# Autodesk Inventor assembly: main assembly
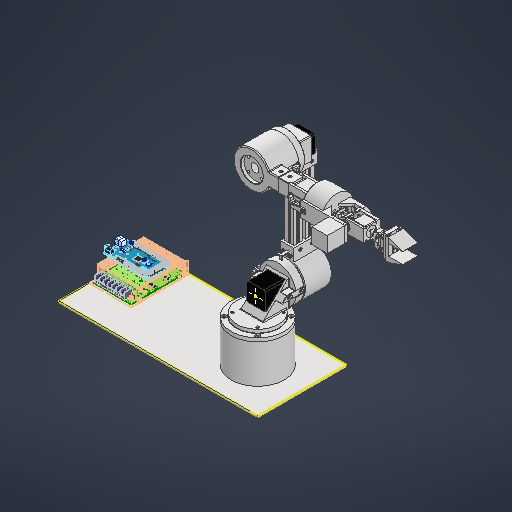
[picture p0: Inventor's stored thumbnail of the model, 512x512]
Saved by Autodesk Inventor 2026.2 (Build 302298000, 298)
## iProperties
Created: 2025-07-04
Part Number: main assembly
Document SubType Name: Assembly
Designer: gavin
Author: gavin
## Documents named in this file (38)
- D:\Github\6-DOF-Robot-Arm\3D-model\robot armT 2(CAD file)\main assembly.iam
- D:\Github\6-DOF-Robot-Arm\3D-model\robot armT 2(CAD file)\stepper 42x48 - 27.ipt
- D:\Github\6-DOF-Robot-Arm\3D-model\robot armT 2(CAD file)\28stepper27.ipt
- D:\Github\6-DOF-Robot-Arm\3D-model\robot armT 2(CAD file)\CSN 02 4630 - 6009.ipt
- D:\Github\6-DOF-Robot-Arm\3D-model\robot armT 2(CAD file)\CNS 2862 B2116 - 6007 - 35 x 62 x 14.ipt
- D:\Github\6-DOF-Robot-Arm\3D-model\robot armT 2(CAD file)\base plate.ipt
- D:\Github\6-DOF-Robot-Arm\3D-model\robot armT 2(CAD file)\stepper 42x60 -50 .ipt
- D:\Github\6-DOF-Robot-Arm\3D-model\robot armT 2(CAD file)\j2 42 motor mount.ipt
- D:\Github\6-DOF-Robot-Arm\3D-model\robot armT 2(CAD file)\j1 assmble.iam
- D:\Github\6-DOF-Robot-Arm\3D-model\robot armT 2(CAD file)\optic endstop module.ipt
- D:\Github\6-DOF-Robot-Arm\3D-model\robot armT 2(CAD file)\j2j3 alumi ext.ipt
- D:\Github\6-DOF-Robot-Arm\3D-model\robot armT 2(CAD file)\j3 motor mount.ipt
- D:\Github\6-DOF-Robot-Arm\3D-model\robot armT 2(CAD file)\j3j4 alumi ext.ipt
- D:\Github\6-DOF-Robot-Arm\3D-model\robot armT 2(CAD file)\j2 endstop blocker.ipt
- D:\Github\6-DOF-Robot-Arm\3D-model\robot armT 2(CAD file)\j3 endstop blocker.ipt
- D:\Github\6-DOF-Robot-Arm\3D-model\robot armT 2(CAD file)\6mm axle hub.ipt
- D:\Github\6-DOF-Robot-Arm\3D-model\robot armT 2(CAD file)\j4 motor mount.ipt
- D:\Github\6-DOF-Robot-Arm\3D-model\robot armT 2(CAD file)\j4 motor mount cover.ipt
- D:\Github\6-DOF-Robot-Arm\3D-model\robot armT 2(CAD file)\j4 moving part.ipt
- D:\Github\6-DOF-Robot-Arm\3D-model\robot armT 2(CAD file)\nema 11x25.ipt
- D:\Github\6-DOF-Robot-Arm\3D-model\robot armT 2(CAD file)\5mm axle hub.ipt
- D:\Github\6-DOF-Robot-Arm\3D-model\robot armT 2(CAD file)\bearing 22-M6.ipt
- D:\Github\6-DOF-Robot-Arm\3D-model\robot armT 2(CAD file)\j6 motor mount v2.ipt
- D:\Github\6-DOF-Robot-Arm\3D-model\robot armT 2(CAD file)\j4 endstop blocker.ipt
- D:\Github\6-DOF-Robot-Arm\3D-model\robot armT 2(CAD file)\sg90 long claw.iam
- D:\Github\6-DOF-Robot-Arm\3D-model\robot armT 2(CAD file)\35x40 stepper.ipt
- D:\Github\6-DOF-Robot-Arm\3D-model\robot armT 2(CAD file)\j3 moving part option3.ipt
- D:\Github\6-DOF-Robot-Arm\3D-model\robot armT 2(CAD file)\z21 8x18.ipt
- D:\Github\6-DOF-Robot-Arm\3D-model\robot armT 2(CAD file)\18mm hub.ipt
- D:\Github\6-DOF-Robot-Arm\3D-model\robot armT 2(CAD file)\j2 moving part option2.ipt
- D:\Github\6-DOF-Robot-Arm\3D-model\robot armT 2(CAD file)\M5 heat set inserts.ipt
- D:\Github\6-DOF-Robot-Arm\3D-model\robot armT 2(CAD file)\AS 1427 - M3 x 6(5) II.ipt
- D:\Github\6-DOF-Robot-Arm\3D-model\robot armT 2(CAD file)\M3 heat set insert.ipt
- D:\Github\6-DOF-Robot-Arm\3D-model\robot armT 2(CAD file)\CNS 4557 - M4 x 0.7 x 10.ipt
- D:\Github\6-DOF-Robot-Arm\3D-model\robot armT 2(CAD file)\AS 1474 - M4(1).ipt
- D:\Github\6-DOF-Robot-Arm\3D-model\robot armT 2(CAD file)\AS 1474 - M3(1).ipt
- D:\Github\6-DOF-Robot-Arm\3D-model\robot armT 2(CAD file)\ArduinoMega2560\ArduinoMega2560\ArduinoMega2560.ipt
- D:\Github\6-DOF-Robot-Arm\3D-model\robot armT 2(CAD file)\VTX-212-100-0xx\VTX-212-100-0xx\VTX-212-100-0xx.ipt
## Components (101 placed, 37 different names)
1. base plate:1 — 齊平:5, 貼合:133, 齊平:22, 貼合:134
2. j1 assmble:1 [sub-assembly]
3. stepper 42x48 - 27:2 — 貼合:45, 貼合:46, 貼合:47, 貼合:110, 齊平:18
4. CSN 02 4630 - 6009:1 — 貼合:48, 貼合:49
5. CSN 02 4630 - 6009:2 — 貼合:16, 貼合:29
6. CNS 2862 B2116 - 6007 - 35 x 62 x 14:1 — 剛性:108, 剛性:109
7. stepper 42x60 -50 :1 — 貼合:16, 貼合:27, 貼合:28, 剛性:106
8. j2 42 motor mount:1 — 貼合:27, 貼合:28, 貼合:29, 貼合:33, 貼合:34, 貼合:35, 剛性:12, 剛性:13
9. optic endstop module:1 — 貼合:33, 貼合:34, 貼合:35, 齊平:10, 剛性:10, 剛性:11
10. j2j3 alumi ext:1 — 剛性:5, 剛性:7
11. j2j3 alumi ext:2 — 剛性:6
12. j3 motor mount:1 — 貼合:45, 貼合:46, 貼合:47, 貼合:48, 貼合:49, 齊平:11, 齊平:12, 貼合:59, 剛性:7, 貼合:132, 剛性:65, 剛性:66, 剛性:67, 剛性:68, 剛性:107
13. j3j4 alumi ext:1 — 剛性:4, 剛性:8
14. optic endstop module:2 — 貼合:129, 貼合:130, 貼合:131, 剛性:20, 剛性:21, 剛性:22, 剛性:23
15. j2 endstop blocker:1 — 齊平:10, 貼合:117, 貼合:118, 貼合:119, 剛性:14, 剛性:15, 剛性:16, 剛性:17
16. j3 endstop blocker:1 — 齊平:11, 齊平:12, 貼合:59, 貼合:132, 剛性:18, 剛性:19, 剛性:24, 剛性:25
17. 6mm axle hub:1 — 貼合:123, 貼合:124, 貼合:125
18. j4 motor mount:1 — 齊平:14, 齊平:15, 貼合:62, 貼合:65, 貼合:71, 貼合:72, 貼合:73, 齊平:21, 剛性:8, 剛性:9, 剛性:27, 剛性:28, 剛性:72, 剛性:75, 剛性:108
19. j4 motor mount cover:1 — 齊平:14, 齊平:15, 貼合:62, 貼合:65
20. 28stepper27:1 — 剛性:9
21. optic endstop module:3 — 貼合:71, 貼合:72, 貼合:73, 剛性:29, 剛性:30
22. j4 moving part:1 — 貼合:74, 貼合:76, 貼合:86, 貼合:87, 貼合:104, 貼合:105, 貼合:107, 貼合:108, 貼合:109, 貼合:123, 貼合:124, 貼合:125, 貼合:126, 貼合:127, 剛性:26, 剛性:32, 剛性:33, 剛性:109
23. nema 11x25:1 — 貼合:88, 貼合:89, 貼合:103, 貼合:128, 剛性:111
24. optic endstop module:4 — 貼合:74, 貼合:76, 貼合:107, 剛性:34, 剛性:35
25. 5mm axle hub:1 — 剛性:1, 剛性:110
26. bearing 22-M6:1 — 貼合:86, 貼合:87
27. j6 motor mount v2:1 — 貼合:88, 貼合:89, 貼合:128, 剛性:110
28. j4 endstop blocker:1 — 貼合:108, 貼合:109, 貼合:126, 剛性:31
29. sg90 long claw:1 [sub-assembly] — 貼合:99, 貼合:100, 貼合:103
30. 5mm axle hub:2 — 貼合:99, 貼合:100, 剛性:111
31. 35x40 stepper:1 — 貼合:104, 貼合:105, 剛性:1, 貼合:127
32. j3 moving part option3:1 — 剛性:4, 貼合:120, 貼合:121, 貼合:122, 齊平:21, 貼合:129, 貼合:130, 貼合:131, 剛性:40, 剛性:41, 剛性:42, 剛性:43, 剛性:73, 剛性:74, 剛性:107
33. z21 8x18:1 — 貼合:110, 齊平:18
34. 18mm hub:1 — 貼合:120, 貼合:121, 貼合:122
35. j2 moving part option2:1 — 剛性:5, 貼合:114, 貼合:115, 貼合:116, 貼合:117, 貼合:118, 貼合:119, 剛性:6, 剛性:36, 剛性:37, 剛性:38, 剛性:39, 剛性:59, 剛性:60, 剛性:61, 剛性:62
36. z21 8x18:2 — 剛性:105, 剛性:106
37. 18mm hub:2 — 剛性:105, 貼合:114, 貼合:115, 貼合:116
38. AS 1427 - M3 x 6(5) II:1 — 剛性:16
39. AS 1427 - M3 x 6(5) II:2 — 剛性:23
40. AS 1427 - M3 x 6(5) II:3 — 剛性:24
41. AS 1427 - M3 x 6(5) II:4 — 剛性:22
42. AS 1427 - M3 x 6(5) II:5 — 剛性:17
43. AS 1427 - M3 x 6(5) II:6 — 剛性:25
44. AS 1427 - M3 x 6(5) II:7 — 剛性:10
45. AS 1427 - M3 x 6(5) II:8 — 剛性:11
46. M3 heat set insert:1 — 剛性:15
47. M3 heat set insert:2 — 剛性:13
48. M3 heat set insert:3 — 剛性:26
49. M3 heat set insert:4 — 剛性:32
50. M3 heat set insert:5 — 剛性:28
51. M3 heat set insert:6 — 剛性:19
52. M3 heat set insert:7 — 剛性:20
53. M3 heat set insert:8 — 剛性:12
54. M3 heat set insert:9 — 剛性:14
55. M3 heat set insert:10 — 剛性:33
56. M3 heat set insert:14 — 剛性:27
57. M3 heat set insert:15 — 剛性:18
58. M3 heat set insert:18 — 剛性:21
59. AS 1427 - M3 x 6(5) II:9 — 剛性:29
60. AS 1427 - M3 x 6(5) II:10 — 剛性:35
61. AS 1427 - M3 x 6(5) II:11 — 剛性:31
62. AS 1427 - M3 x 6(5) II:12 — 剛性:30
63. AS 1427 - M3 x 6(5) II:13 — 剛性:34
64. M5 heat set inserts:5 — 剛性:39
65. M5 heat set inserts:6 — 剛性:36
66. M5 heat set inserts:10 — 剛性:42
67. M5 heat set inserts:11 — 剛性:41
68. M5 heat set inserts:12 — 剛性:40
69. M5 heat set inserts:13 — 剛性:38
70. M5 heat set inserts:14 — 剛性:37
71. M5 heat set inserts:18 — 剛性:43
72. CNS 4557 - M4 x 0.7 x 10:1 — 剛性:64, 剛性:65
73. CNS 4557 - M4 x 0.7 x 10:2 — 剛性:57, 剛性:60
74. CNS 4557 - M4 x 0.7 x 10:3 — 剛性:55, 剛性:74
75. CNS 4557 - M4 x 0.7 x 10:4 — 剛性:53, 剛性:67
76. CNS 4557 - M4 x 0.7 x 10:5 — 剛性:58, 剛性:59
77. CNS 4557 - M4 x 0.7 x 10:6 — 剛性:56, 剛性:62
78. CNS 4557 - M4 x 0.7 x 10:7 — 剛性:54, 剛性:68
79. CNS 4557 - M4 x 0.7 x 10:8 — 剛性:52, 剛性:61
80. CNS 4557 - M4 x 0.7 x 10:9 — 剛性:71, 剛性:72
81. CNS 4557 - M4 x 0.7 x 10:10 — 剛性:70, 剛性:73
82. CNS 4557 - M4 x 0.7 x 10:11 — 剛性:63, 剛性:66
83. CNS 4557 - M4 x 0.7 x 10:12 — 剛性:69, 剛性:75
84. AS 1474 - M4(1):1 — 剛性:57
85. AS 1474 - M4(1):2 — 剛性:55
86. AS 1474 - M4(1):5 — 剛性:56
87. AS 1474 - M4(1):6 — 剛性:53
88. AS 1474 - M4(1):7 — 剛性:54
89. AS 1474 - M4(1):11 — 剛性:64
90. AS 1474 - M4(1):12 — 剛性:63
91. AS 1474 - M4(1):13 — 剛性:71
92. AS 1474 - M4(1):14 — 剛性:69
93. AS 1474 - M4(1):15 — 剛性:70
94. AS 1474 - M4(1):16 — 剛性:52
95. AS 1474 - M4(1):18 — 剛性:58
96. AS 1474 - M3(1):1
97. AS 1474 - M3(1):2
98. AS 1474 - M3(1):3
99. AS 1474 - M3(1):5
100. ArduinoMega2560:1
101. VTX-212-100-0xx:1 — 貼合:133, 齊平:22, 貼合:134
## Relationships (149: WeldJoint 72, Mate 61, Flush 10, RevoluteJoint 6)
- [Mate]: j1 assmble:1
- [Flush]: base plate:1 ↔ j1 assmble:1
- [Mate]: base plate:1 ↔ j1 assmble:1
- 齊平:5 [Flush]: base plate:1
- 貼合:16 [Mate]: CSN 02 4630 - 6009:2 ↔ stepper 42x60 -50 :1
- [Mate] (20 mm): j1 assmble:1 ↔ stepper 42x60 -50 :1
- [Mate]: j1 assmble:1 ↔ j2 42 motor mount:1
- [Mate]: base plate:1 ↔ j1 assmble:1
- [Mate]: j1 assmble:1 ↔ j2 42 motor mount:1
- [Mate]: j1 assmble:1 ↔ j2 42 motor mount:1
- 貼合:27 [Mate]: stepper 42x60 -50 :1 ↔ j2 42 motor mount:1
- 貼合:28 [Mate]: stepper 42x60 -50 :1 ↔ j2 42 motor mount:1
- 貼合:29 [Mate]: CSN 02 4630 - 6009:2 ↔ j2 42 motor mount:1
- [RevoluteJoint]: base plate:1 ↔ j1 assmble:1
- [RevoluteJoint]: base plate:1 ↔ j1 assmble:1
- [RevoluteJoint]: base plate:1 ↔ j1 assmble:1
- [RevoluteJoint]: base plate:1 ↔ j1 assmble:1
- [RevoluteJoint]: base plate:1 ↔ j1 assmble:1
- [RevoluteJoint]: base plate:1 ↔ j1 assmble:1
- 貼合:33 [Mate]: j2 42 motor mount:1 ↔ optic endstop module:1
- 貼合:34 [Mate]: j2 42 motor mount:1 ↔ optic endstop module:1
- 貼合:35 [Mate]: j2 42 motor mount:1 ↔ optic endstop module:1
- 貼合:45 [Mate]: stepper 42x48 - 27:2 ↔ j3 motor mount:1
- 貼合:46 [Mate] (0.075 mm): stepper 42x48 - 27:2 ↔ j3 motor mount:1
- 貼合:47 [Mate]: stepper 42x48 - 27:2 ↔ j3 motor mount:1
- 貼合:48 [Mate]: CSN 02 4630 - 6009:1 ↔ j3 motor mount:1
- 貼合:49 [Mate]: CSN 02 4630 - 6009:1 ↔ j3 motor mount:1
- 齊平:10 [Flush]: optic endstop module:1 ↔ j2 endstop blocker:1
- 齊平:11 [Flush]: j3 motor mount:1 ↔ j3 endstop blocker:1
- 齊平:12 [Flush]: j3 motor mount:1 ↔ j3 endstop blocker:1
- 齊平:14 [Flush]: j4 motor mount:1 ↔ j4 motor mount cover:1
- 齊平:15 [Flush]: j4 motor mount:1 ↔ j4 motor mount cover:1
- 貼合:59 [Mate]: j3 motor mount:1 ↔ j3 endstop blocker:1
- 貼合:62 [Mate]: j4 motor mount:1 ↔ j4 motor mount cover:1
- 貼合:65 [Mate]: j4 motor mount:1 ↔ j4 motor mount cover:1
- 貼合:71 [Mate]: j4 motor mount:1 ↔ optic endstop module:3
- 貼合:72 [Mate]: j4 motor mount:1 ↔ optic endstop module:3
- 貼合:73 [Mate]: j4 motor mount:1 ↔ optic endstop module:3
- 貼合:74 [Mate]: j4 moving part:1 ↔ optic endstop module:4
- 貼合:76 [Mate]: j4 moving part:1 ↔ optic endstop module:4
- 貼合:86 [Mate]: j4 moving part:1 ↔ bearing 22-M6:1
- 貼合:87 [Mate]: j4 moving part:1 ↔ bearing 22-M6:1
- 貼合:88 [Mate]: nema 11x25:1 ↔ j6 motor mount v2:1
- 貼合:89 [Mate]: nema 11x25:1 ↔ j6 motor mount v2:1
- 貼合:99 [Mate]: sg90 long claw:1 ↔ 5mm axle hub:2
- 貼合:100 [Mate]: sg90 long claw:1 ↔ 5mm axle hub:2
- 貼合:103 [Mate]: nema 11x25:1 ↔ sg90 long claw:1
- 貼合:104 [Mate]: j4 moving part:1 ↔ 35x40 stepper:1
- 貼合:105 [Mate]: j4 moving part:1 ↔ 35x40 stepper:1
- 剛性:1 [WeldJoint]: 5mm axle hub:1 ↔ 35x40 stepper:1
- 貼合:107 [Mate]: j4 moving part:1 ↔ optic endstop module:4
- 貼合:108 [Mate]: j4 moving part:1 ↔ j4 endstop blocker:1
- 貼合:109 [Mate]: j4 moving part:1 ↔ j4 endstop blocker:1
- 貼合:110 [Mate]: stepper 42x48 - 27:2 ↔ z21 8x18:1
- 齊平:18 [Flush]: stepper 42x48 - 27:2 ↔ z21 8x18:1
- 剛性:105 [WeldJoint] (-3.71 mm): z21 8x18:2 ↔ 18mm hub:2
- 剛性:4 [WeldJoint]: j3j4 alumi ext:1 ↔ j3 moving part option3:1
- 剛性:5 [WeldJoint]: j2j3 alumi ext:1 ↔ j2 moving part option2:1
- 貼合:114 [Mate]: j2 moving part option2:1 ↔ 18mm hub:2
- 貼合:115 [Mate]: j2 moving part option2:1 ↔ 18mm hub:2
- 貼合:116 [Mate]: j2 moving part option2:1 ↔ 18mm hub:2
- 貼合:117 [Mate]: j2 endstop blocker:1 ↔ j2 moving part option2:1
- 貼合:118 [Mate]: j2 endstop blocker:1 ↔ j2 moving part option2:1
- 貼合:119 [Mate]: j2 endstop blocker:1 ↔ j2 moving part option2:1
- 剛性:6 [WeldJoint]: j2j3 alumi ext:2 ↔ j2 moving part option2:1
- 剛性:7 [WeldJoint]: j2j3 alumi ext:1 ↔ j3 motor mount:1
- 貼合:120 [Mate]: j3 moving part option3:1 ↔ 18mm hub:1
- 貼合:121 [Mate]: j3 moving part option3:1 ↔ 18mm hub:1
- 貼合:122 [Mate]: j3 moving part option3:1 ↔ 18mm hub:1
- 齊平:21 [Flush]: j4 motor mount:1 ↔ j3 moving part option3:1
- 剛性:8 [WeldJoint]: j3j4 alumi ext:1 ↔ j4 motor mount:1
- 剛性:9 [WeldJoint]: j4 motor mount:1 ↔ 28stepper27:1
- 貼合:123 [Mate]: 6mm axle hub:1 ↔ j4 moving part:1
- 貼合:124 [Mate]: 6mm axle hub:1 ↔ j4 moving part:1
- 貼合:125 [Mate]: 6mm axle hub:1 ↔ j4 moving part:1
- 貼合:126 [Mate]: j4 moving part:1 ↔ j4 endstop blocker:1
- 貼合:127 [Mate]: j4 moving part:1 ↔ 35x40 stepper:1
- 貼合:128 [Mate]: nema 11x25:1 ↔ j6 motor mount v2:1
- 貼合:129 [Mate]: optic endstop module:2 ↔ j3 moving part option3:1
- 貼合:130 [Mate]: optic endstop module:2 ↔ j3 moving part option3:1
- 貼合:131 [Mate]: optic endstop module:2 ↔ j3 moving part option3:1
- 貼合:132 [Mate]: j3 motor mount:1 ↔ j3 endstop blocker:1
- 剛性:10 [WeldJoint]: optic endstop module:1 ↔ AS 1427 - M3 x 6(5) II:7
- 剛性:11 [WeldJoint]: optic endstop module:1 ↔ AS 1427 - M3 x 6(5) II:8
- 剛性:12 [WeldJoint]: j2 42 motor mount:1 ↔ M3 heat set insert:8
- 剛性:13 [WeldJoint]: j2 42 motor mount:1 ↔ M3 heat set insert:2
- 剛性:14 [WeldJoint]: j2 endstop blocker:1 ↔ M3 heat set insert:9
- 剛性:15 [WeldJoint]: j2 endstop blocker:1 ↔ M3 heat set insert:1
- 剛性:16 [WeldJoint]: j2 endstop blocker:1 ↔ AS 1427 - M3 x 6(5) II:1
- 剛性:17 [WeldJoint]: j2 endstop blocker:1 ↔ AS 1427 - M3 x 6(5) II:5
- 剛性:18 [WeldJoint]: j3 endstop blocker:1 ↔ M3 heat set insert:15
- 剛性:19 [WeldJoint]: j3 endstop blocker:1 ↔ M3 heat set insert:6
- 剛性:20 [WeldJoint]: optic endstop module:2 ↔ M3 heat set insert:7
- 剛性:21 [WeldJoint]: optic endstop module:2 ↔ M3 heat set insert:18
- 剛性:22 [WeldJoint]: optic endstop module:2 ↔ AS 1427 - M3 x 6(5) II:4
- 剛性:23 [WeldJoint]: optic endstop module:2 ↔ AS 1427 - M3 x 6(5) II:2
- 剛性:24 [WeldJoint]: j3 endstop blocker:1 ↔ AS 1427 - M3 x 6(5) II:3
- 剛性:25 [WeldJoint]: j3 endstop blocker:1 ↔ AS 1427 - M3 x 6(5) II:6
- 剛性:26 [WeldJoint]: j4 moving part:1 ↔ M3 heat set insert:3
- 剛性:27 [WeldJoint]: j4 motor mount:1 ↔ M3 heat set insert:14
- 剛性:28 [WeldJoint]: j4 motor mount:1 ↔ M3 heat set insert:5
- 剛性:29 [WeldJoint]: optic endstop module:3 ↔ AS 1427 - M3 x 6(5) II:9
- 剛性:30 [WeldJoint]: optic endstop module:3 ↔ AS 1427 - M3 x 6(5) II:12
- 剛性:31 [WeldJoint]: j4 endstop blocker:1 ↔ AS 1427 - M3 x 6(5) II:11
- 剛性:32 [WeldJoint]: j4 moving part:1 ↔ M3 heat set insert:4
- 剛性:33 [WeldJoint]: j4 moving part:1 ↔ M3 heat set insert:10
- 剛性:34 [WeldJoint]: optic endstop module:4 ↔ AS 1427 - M3 x 6(5) II:13
- 剛性:35 [WeldJoint]: optic endstop module:4 ↔ AS 1427 - M3 x 6(5) II:10
- 剛性:36 [WeldJoint]: j2 moving part option2:1 ↔ M5 heat set inserts:6
- 剛性:37 [WeldJoint]: j2 moving part option2:1 ↔ M5 heat set inserts:14
- 剛性:38 [WeldJoint]: j2 moving part option2:1 ↔ M5 heat set inserts:13
- 剛性:39 [WeldJoint]: j2 moving part option2:1 ↔ M5 heat set inserts:5
- 剛性:40 [WeldJoint]: j3 moving part option3:1 ↔ M5 heat set inserts:12
- 剛性:41 [WeldJoint]: j3 moving part option3:1 ↔ M5 heat set inserts:11
- 剛性:42 [WeldJoint]: j3 moving part option3:1 ↔ M5 heat set inserts:10
- 剛性:43 [WeldJoint]: j3 moving part option3:1 ↔ M5 heat set inserts:18
- 剛性:52 [WeldJoint] (10 mm): CNS 4557 - M4 x 0.7 x 10:8 ↔ AS 1474 - M4(1):16
- 剛性:53 [WeldJoint]: CNS 4557 - M4 x 0.7 x 10:4 ↔ AS 1474 - M4(1):6
- 剛性:54 [WeldJoint]: CNS 4557 - M4 x 0.7 x 10:7 ↔ AS 1474 - M4(1):7
- 剛性:55 [WeldJoint]: CNS 4557 - M4 x 0.7 x 10:3 ↔ AS 1474 - M4(1):2
- 剛性:56 [WeldJoint]: CNS 4557 - M4 x 0.7 x 10:6 ↔ AS 1474 - M4(1):5
- 剛性:57 [WeldJoint]: CNS 4557 - M4 x 0.7 x 10:2 ↔ AS 1474 - M4(1):1
- 剛性:58 [WeldJoint]: CNS 4557 - M4 x 0.7 x 10:5 ↔ AS 1474 - M4(1):18
- 剛性:59 [WeldJoint]: j2 moving part option2:1 ↔ CNS 4557 - M4 x 0.7 x 10:5
- 剛性:60 [WeldJoint]: j2 moving part option2:1 ↔ CNS 4557 - M4 x 0.7 x 10:2
- 剛性:61 [WeldJoint]: j2 moving part option2:1 ↔ CNS 4557 - M4 x 0.7 x 10:8
- 剛性:62 [WeldJoint]: j2 moving part option2:1 ↔ CNS 4557 - M4 x 0.7 x 10:6
- 剛性:63 [WeldJoint]: CNS 4557 - M4 x 0.7 x 10:11 ↔ AS 1474 - M4(1):12
- 剛性:64 [WeldJoint]: CNS 4557 - M4 x 0.7 x 10:1 ↔ AS 1474 - M4(1):11
- 剛性:65 [WeldJoint]: j3 motor mount:1 ↔ CNS 4557 - M4 x 0.7 x 10:1
- 剛性:66 [WeldJoint]: j3 motor mount:1 ↔ CNS 4557 - M4 x 0.7 x 10:11
- 剛性:67 [WeldJoint]: j3 motor mount:1 ↔ CNS 4557 - M4 x 0.7 x 10:4
- 剛性:68 [WeldJoint]: j3 motor mount:1 ↔ CNS 4557 - M4 x 0.7 x 10:7
- 剛性:69 [WeldJoint]: CNS 4557 - M4 x 0.7 x 10:12 ↔ AS 1474 - M4(1):14
- 剛性:70 [WeldJoint]: CNS 4557 - M4 x 0.7 x 10:10 ↔ AS 1474 - M4(1):15
- 剛性:71 [WeldJoint]: CNS 4557 - M4 x 0.7 x 10:9 ↔ AS 1474 - M4(1):13
- 剛性:72 [WeldJoint]: j4 motor mount:1 ↔ CNS 4557 - M4 x 0.7 x 10:9
- 剛性:73 [WeldJoint]: j3 moving part option3:1 ↔ CNS 4557 - M4 x 0.7 x 10:10
- 剛性:74 [WeldJoint]: j3 moving part option3:1 ↔ CNS 4557 - M4 x 0.7 x 10:3
- 剛性:75 [WeldJoint]: j4 motor mount:1 ↔ CNS 4557 - M4 x 0.7 x 10:12
- 剛性:106 [WeldJoint]: stepper 42x60 -50 :1 ↔ z21 8x18:2
- 剛性:107 [WeldJoint]: j3 motor mount:1 ↔ j3 moving part option3:1
- 剛性:108 [WeldJoint]: CNS 2862 B2116 - 6007 - 35 x 62 x 14:1 ↔ j4 motor mount:1
- 剛性:109 [WeldJoint]: CNS 2862 B2116 - 6007 - 35 x 62 x 14:1 ↔ j4 moving part:1
- 剛性:110 [WeldJoint]: 5mm axle hub:1 ↔ j6 motor mount v2:1
- 剛性:111 [WeldJoint]: nema 11x25:1 ↔ 5mm axle hub:2
- 貼合:133 [Mate]: base plate:1 ↔ VTX-212-100-0xx:1
- 齊平:22 [Flush]: base plate:1 ↔ VTX-212-100-0xx:1
- 貼合:134 [Mate] (-3 mm): base plate:1 ↔ VTX-212-100-0xx:1
## Named parameters: d225_d219 = -3.71 mm
